# Autodesk Inventor assembly: 2A.01.01.02.IM.AileronAssembly
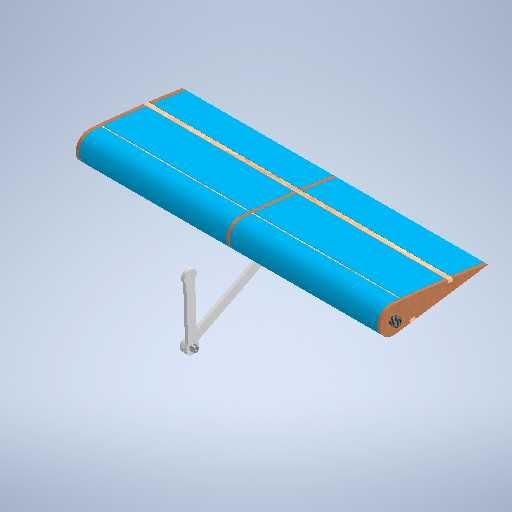
[picture p0: Inventor's stored thumbnail of the model, 512x512]
Saved by Autodesk Inventor 2025.2 (Build 292293000, 293)
## iProperties
Created: 2025-01-27
Part Number: 2A.01.01.02.IM.AileronAssembly
Document SubType Name: Assembly
Designer: Imist
Author: Imist
## Documents named in this file (14)
- C:\Users\Imist\OneDrive - University of Bristol\Year 2\AVDASI 2\Team\Final CAD\2A.01.01.02.IM.AileronAssembly.iam
- C:\Users\Imist\OneDrive - University of Bristol\Year 2\AVDASI 2\Team\Final CAD\2P.03.01.02.IM.AileronBody.ipt
- C:\Users\Imist\OneDrive - University of Bristol\Year 2\AVDASI 2\Team\Final CAD\2P.03.01.03.IM.AileronSpar.ipt
- C:\Users\Imist\OneDrive - University of Bristol\Year 2\AVDASI 2\Team\Final CAD\2P.03.01.06.IM.AileronCutFill.ipt
- C:\Users\Imist\OneDrive - University of Bristol\Year 2\AVDASI 2\Team\Final CAD\2P.03.01.08.JW.AileronRibMid.ipt
- C:\Users\Imist\OneDrive - University of Bristol\Year 2\AVDASI 2\Team\Final CAD\2P.03.01.10.IM.AileronRibEnd.ipt
- C:\Users\Imist\OneDrive - University of Bristol\Year 2\AVDASI 2\Team\Final CAD\2P.03.01.13.IM.AilBottSpanBeam.ipt
- C:\Users\Imist\OneDrive - University of Bristol\Year 2\AVDASI 2\Team\Final CAD\2P.03.01.14.IM.AilTopSpanBeam.ipt
- C:\Users\Imist\OneDrive - University of Bristol\Year 2\AVDASI 2\Team\Final CAD\2P.03.01.17.ZW.AileronCoupler.ipt
- C:\Users\Imist\OneDrive - University of Bristol\Year 2\AVDASI 2\Team\Final CAD\2P.03.01.18.ZW.AileronCrank.ipt
- C:\Users\Imist\OneDrive\Documents\Inventor\Content Center Files\R2025\en-US\ISO 7092\ISO 7092 - ST 3 - 140 HV.ipt
- C:\Users\Imist\OneDrive - University of Bristol\Year 2\AVDASI 2\Team\Final CAD\2P.03.01.00.01.IM.Bearing3x7x3.ipt
- C:\Users\Imist\OneDrive\Documents\Inventor\Content Center Files\R2025\en-US\AS 1420\AS 1420 - 1973 - M3 x 10.ipt
- C:\Users\Imist\OneDrive\Documents\Inventor\Content Center Files\R2025\en-US\AS 1112 (4)\AS 1112 - M3(2).ipt
## Components (26 placed, 13 different names)
1. 2P.03.01.02.IM.AileronBody:1 — Rigid:1, Rigid:3, Rigid:6
2. 2P.03.01.03.IM.AileronSpar:1 — Rigid:9, Mate:1, Mate:2, Mate:3, Mate:4
3. 2P.03.01.06.IM.AileronCutFill:1 — Rigid:1
4. 2P.03.01.08.JW.AileronRibMid:1 — Rigid:3, Rigid:4, Rigid:10
5. 2P.03.01.10.IM.AileronRibEnd:1 — Rigid:5, Rigid:7, Rigid:8, Rigid:9
6. 2P.03.01.13.IM.AilBottSpanBeam:1 — Rigid:8
7. 2P.03.01.14.IM.AilTopSpanBeam:1 — Rigid:7
8. 2P.03.01.17.ZW.AileronCoupler:1 — Rigid:11, Rigid:12
9. 2P.03.01.18.ZW.AileronCrank:1 — Rigid:13
10. 2P.03.01.02.IM.AileronBody:2 — Rigid:4, Rigid:5
11. 2P.03.01.06.IM.AileronCutFill:2
12. 2P.03.01.10.IM.AileronRibEnd:2 — Rigid:6
13. ISO 7092 ST 3 - 140 HV:1 — Rotational:1, Rotational:2
14. ISO 7092 ST 3 - 140 HV:2 — Rotational:3, Rotational:8
15. ISO 7092 ST 3 - 140 HV:3 — Rotational:10, Rotational:11
16. ISO 7092 ST 3 - 140 HV:4 — Rotational:4, Rotational:7
17. ISO 7092 ST 3 - 140 HV:5 — Rotational:6, Rotational:12
18. ISO 7092 ST 3 - 140 HV:6 — Rotational:5, Rotational:9
19. 2P.03.01.00.01.IM.Bearing3x7x3:1 — Rigid:10, Rotational:1, Rotational:10
20. 2P.03.01.00.01.IM.Bearing3x7x3:2 — Rigid:12, Rotational:4, Rotational:6
21. 2P.03.01.00.01.IM.Bearing3x7x3:3 — Rigid:11, Rotational:2, Rotational:3
22. 2P.03.01.00.01.IM.Bearing3x7x3:4 — Rigid:13, Rotational:5, Rotational:7
23. AS 1420 - Metric M3 x 10:1 — Rotational:8
24. AS 1420 - Metric M3 x 10:2 — Rotational:9
25. AS 1112 (4) - Metric M3:1 — Rotational:12
26. AS 1112 (4) - Metric M3:2 — Rotational:11
## Relationships (29: WeldJoint 13, RevoluteJoint 12, Mate 4)
- Rigid:1 [WeldJoint]: 2P.03.01.02.IM.AileronBody:1 ↔ 2P.03.01.06.IM.AileronCutFill:1
- [WeldJoint]: 2P.03.01.02.IM.AileronBody:2 ↔ 2P.03.01.06.IM.AileronCutFill:2
- Rigid:3 [WeldJoint]: 2P.03.01.02.IM.AileronBody:1 ↔ 2P.03.01.08.JW.AileronRibMid:1
- Rigid:4 [WeldJoint]: 2P.03.01.08.JW.AileronRibMid:1 ↔ 2P.03.01.02.IM.AileronBody:2
- Rigid:5 [WeldJoint]: 2P.03.01.10.IM.AileronRibEnd:1 ↔ 2P.03.01.02.IM.AileronBody:2
- Rigid:6 [WeldJoint]: 2P.03.01.02.IM.AileronBody:1 ↔ 2P.03.01.10.IM.AileronRibEnd:2
- Rigid:7 [WeldJoint]: 2P.03.01.10.IM.AileronRibEnd:1 ↔ 2P.03.01.14.IM.AilTopSpanBeam:1
- Rigid:8 [WeldJoint]: 2P.03.01.10.IM.AileronRibEnd:1 ↔ 2P.03.01.13.IM.AilBottSpanBeam:1
- Rigid:9 [WeldJoint] (-4.5 mm): 2P.03.01.03.IM.AileronSpar:1 ↔ 2P.03.01.10.IM.AileronRibEnd:1
- Rigid:10 [WeldJoint]: 2P.03.01.08.JW.AileronRibMid:1 ↔ 2P.03.01.00.01.IM.Bearing3x7x3:1
- Rotational:1 [RevoluteJoint] (-0.5 mm): ISO 7092 ST 3 - 140 HV:1 ↔ 2P.03.01.00.01.IM.Bearing3x7x3:1
- Rigid:11 [WeldJoint]: 2P.03.01.17.ZW.AileronCoupler:1 ↔ 2P.03.01.00.01.IM.Bearing3x7x3:3
- Rotational:2 [RevoluteJoint]: ISO 7092 ST 3 - 140 HV:1 ↔ 2P.03.01.00.01.IM.Bearing3x7x3:3
- Rotational:3 [RevoluteJoint] (0.5 mm): ISO 7092 ST 3 - 140 HV:2 ↔ 2P.03.01.00.01.IM.Bearing3x7x3:3
- Rigid:12 [WeldJoint]: 2P.03.01.17.ZW.AileronCoupler:1 ↔ 2P.03.01.00.01.IM.Bearing3x7x3:2
- Rigid:13 [WeldJoint]: 2P.03.01.18.ZW.AileronCrank:1 ↔ 2P.03.01.00.01.IM.Bearing3x7x3:4
- Rotational:4 [RevoluteJoint] (0.5 mm): ISO 7092 ST 3 - 140 HV:4 ↔ 2P.03.01.00.01.IM.Bearing3x7x3:2
- Rotational:5 [RevoluteJoint] (0.5 mm): ISO 7092 ST 3 - 140 HV:6 ↔ 2P.03.01.00.01.IM.Bearing3x7x3:4
- Rotational:6 [RevoluteJoint]: ISO 7092 ST 3 - 140 HV:5 ↔ 2P.03.01.00.01.IM.Bearing3x7x3:2
- Rotational:7 [RevoluteJoint]: ISO 7092 ST 3 - 140 HV:4 ↔ 2P.03.01.00.01.IM.Bearing3x7x3:4
- Rotational:8 [RevoluteJoint]: ISO 7092 ST 3 - 140 HV:2 ↔ AS 1420 - Metric M3 x 10:1
- Rotational:9 [RevoluteJoint]: ISO 7092 ST 3 - 140 HV:6 ↔ AS 1420 - Metric M3 x 10:2
- Rotational:10 [RevoluteJoint] (-0.5 mm): ISO 7092 ST 3 - 140 HV:3 ↔ 2P.03.01.00.01.IM.Bearing3x7x3:1
- Rotational:11 [RevoluteJoint]: ISO 7092 ST 3 - 140 HV:3 ↔ AS 1112 (4) - Metric M3:2
- Rotational:12 [RevoluteJoint]: ISO 7092 ST 3 - 140 HV:5 ↔ AS 1112 (4) - Metric M3:1
- Mate:1: 2P.03.01.03.IM.AileronSpar:1
- Mate:2: 2P.03.01.03.IM.AileronSpar:1
- Mate:3: 2P.03.01.03.IM.AileronSpar:1
- Mate:4: 2P.03.01.03.IM.AileronSpar:1
## Named parameters: d1_d0 = 0 mm
